# Autodesk Inventor assembly: Сборка стойка
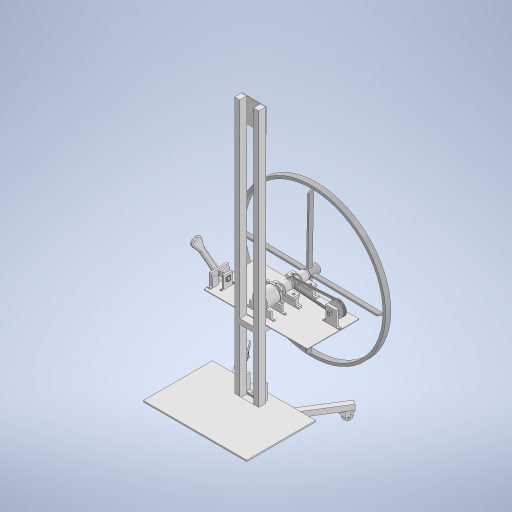
[picture p0: Inventor's stored thumbnail of the model, 512x512]
Saved by Autodesk Inventor 2023 (Build 270158000, 158)
## iProperties
Created: 2022-05-29
Part Number: Сборка стойка
Document SubType Name: Assembly
Designer: avkap
Author: avkap
## Documents named in this file (7)
- D:\Стойка\VR-simulator-3D-models\Стойка\Сборка стойка.iam
- D:\Стойка\VR-simulator-3D-models\Стойка\Стойка.ipt
- D:\Стойка\VR-simulator-3D-models\Механизм\Сборка штурвал.iam
- D:\Стойка\VR-simulator-3D-models\Механизм\Нижняя полка.ipt
- D:\Стойка\VR-simulator-3D-models\Архив\Пластина.ipt
- D:\Стойка\VR-simulator-3D-models\Архив\Колесо.ipt
- D:\Стойка\VR-simulator-3D-models\Механизм\Скоба для полки.ipt
## Components (9 placed, 6 different names)
1. Стойка:1 — Совмещение:3, Заподлицо:2, Совмещение:5, Совмещение:6, Совмещение:7, Совмещение:8, Совмещение:9, Совмещение:10, Заподлицо:4, Заподлицо:5, Заподлицо:6, Заподлицо:7, Заподлицо:8, Заподлицо:9, Заподлицо:10, Заподлицо:11, Совмещение:11, Совмещение:12, Совмещение:13, Заподлицо:12, Совмещение:15, Заподлицо:13
2. Нижняя полка:1 — Совмещение:3, Совмещение:11, Совмещение:12, Совмещение:14
3. Пластина:1 — Заподлицо:2, Совмещение:13, Заподлицо:12
4. Колесо:1 — Совмещение:8, Заподлицо:6, Заподлицо:7
5. Колесо:2 — Совмещение:10, Заподлицо:10, Заподлицо:11
6. Колесо:3 — Совмещение:9, Заподлицо:8, Заподлицо:9
7. Колесо:4 — Совмещение:7, Заподлицо:4, Заподлицо:5
8. Скоба для полки:1 — Совмещение:14, Совмещение:15, Заподлицо:13
9. Сборка штурвал:1 [sub-assembly] — Совмещение:5, Совмещение:6
## Relationships (23: Mate 12, Flush 11)
- Совмещение:3 [Mate]: Стойка:1 ↔ Нижняя полка:1
- Заподлицо:2 [Flush]: Стойка:1 ↔ Пластина:1
- Совмещение:5 [Mate]: Стойка:1 ↔ Сборка штурвал:1
- Совмещение:6 [Mate]: Стойка:1 ↔ Сборка штурвал:1
- Совмещение:7 [Mate]: Стойка:1 ↔ Колесо:4
- Совмещение:8 [Mate]: Стойка:1 ↔ Колесо:1
- Совмещение:9 [Mate]: Стойка:1 ↔ Колесо:3
- Совмещение:10 [Mate]: Стойка:1 ↔ Колесо:2
- Заподлицо:4 [Flush]: Стойка:1 ↔ Колесо:4
- Заподлицо:5 [Flush]: Стойка:1 ↔ Колесо:4
- Заподлицо:6 [Flush]: Стойка:1 ↔ Колесо:1
- Заподлицо:7 [Flush]: Стойка:1 ↔ Колесо:1
- Заподлицо:8 [Flush]: Стойка:1 ↔ Колесо:3
- Заподлицо:9 [Flush]: Стойка:1 ↔ Колесо:3
- Заподлицо:10 [Flush]: Стойка:1 ↔ Колесо:2
- Заподлицо:11 [Flush]: Стойка:1 ↔ Колесо:2
- Совмещение:11 [Mate]: Стойка:1 ↔ Нижняя полка:1
- Совмещение:12 [Mate]: Стойка:1 ↔ Нижняя полка:1
- Совмещение:13 [Mate]: Стойка:1 ↔ Пластина:1
- Заподлицо:12 [Flush]: Стойка:1 ↔ Пластина:1
- Совмещение:14 [Mate]: Нижняя полка:1 ↔ Скоба для полки:1
- Совмещение:15 [Mate]: Стойка:1 ↔ Скоба для полки:1
- Заподлицо:13 [Flush]: Стойка:1 ↔ Скоба для полки:1
